# Autodesk Inventor assembly: ASY NVPH-400 shredder
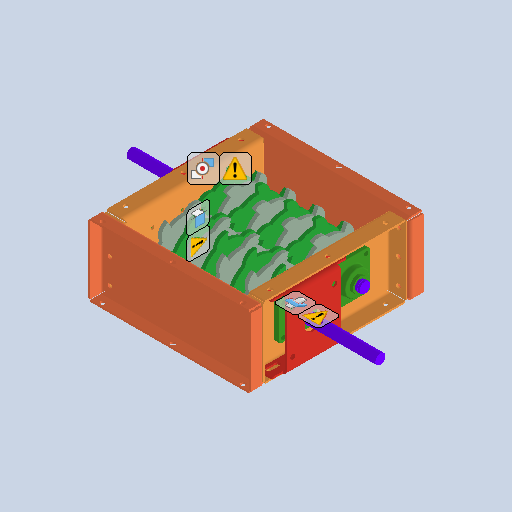
[picture p0: Inventor's stored thumbnail of the model, 512x512]
Saved by Autodesk Inventor 2025 (Build 290162010, 162A)
## iProperties
Created: 2024-12-13
Part Number: ASY NVPH-400 shredder
Document SubType Name: Assembly
Designer: user
Author: user
## Documents named in this file (12)
- C:\Users\pokla\Documents\Inventor\NDM-VOS_powder_hopper\ASY NVPH-400 shredder.iam
- C:\Users\pokla\Documents\Inventor\NDM-VOS_powder_hopper\ASY NVPH-200 shredder shaft full.iam
- C:\Users\pokla\Documents\Inventor\NDM-VOS_powder_hopper\NDM-VOS 111 sredder wall 1.ipt
- C:\Users\pokla\Documents\Inventor\NDM-VOS_powder_hopper\3d party\PCRV080-075SHFA_MS80B5\PCRV080-075SHFA_MS80B5\PCRV080-075SHFA_MS80B5.ipt
- C:\Users\pokla\Documents\Inventor\NDM-VOS_powder_hopper\NDM-VOS 112 sredder wall 2.ipt
- C:\Users\pokla\Documents\Inventor\NDM-VOS_powder_hopper\NDM-VOS dummy Disc Harrow Pillow block bearing mount Assembly.ipt
- C:\Users\DELL\YandexDisk-badmisterfox\домашниий пк\Inventor\Content Center Files\en-US\ISO 4017(1)\ISO 4017 - M12 x 35 - ISO.ipt
- C:\Users\pokla\Documents\Inventor\NDM-VOS_powder_hopper\NDM-VOS 116 engine plate.ipt
- C:\Users\DELL\YandexDisk-badmisterfox\домашниий пк\Inventor\Content Center Files\en-US\ISO 4017(1)\ISO 4017 - M12 x 40 - ISO.ipt
- C:\Users\pokla\Documents\Inventor\NDM-VOS_powder_hopper\NDM-VOS 161 harrow plate.ipt
- C:\Users\pokla\Documents\Inventor\NDM-VOS_powder_hopper\NDM-VOS 162 harrow plate 5.ipt
- C:\Users\DELL\YandexDisk-badmisterfox\домашниий пк\Inventor\Content Center Files\en-US\ISO 4017(1)\ISO 4017 - M12 x 25 - ISO.ipt
## Components (60 placed, 11 different names)
1. ASY NVPH-200 shredder shaft full:1 [sub-assembly] — Rotational:1, Mate:3
2. ASY NVPH-200 shredder shaft full:2 [sub-assembly] — Rotational:2, Mate:4
3. NDM-VOS 111 sredder wall 1:1 — Rigid:1, Rigid:3, Insert:13, Insert:14, Insert:15, Insert:17, Flush:1, Rigid:6, Rigid:7, Rotational:1, Rotational:13, Rotational:14, Slider:2, Rotational:15, Rotational:16
4. NDM-VOS 111 sredder wall 1:2 — Rigid:2, Insert:20, Insert:22, Insert:23, Insert:24, Rigid:8, Rigid:11, Rotational:2, Rotational:11, Rigid:12, Rigid:13, Rigid:14, Rigid:15, Rigid:16, Rigid:17, Rigid:18, Slider:1, Rigid:19, Rotational:12
5. PCRV080-075SHFA_MS80B5:1 — Rotational:17
6. PCRV080-075SHFA_MS80B5:2 — Rigid:20
7. NDM-VOS 112 sredder wall sub:1 — Rigid:1, Rigid:2, Insert:1, Insert:2, Insert:3, Insert:4, Insert:5, Insert:6, Insert:7, Insert:8, Insert:9, Insert:10, Insert:11, Insert:12, Mate:1, Mate:2
8. NDM-VOS 112 sredder wall sub:2 — Rigid:3, Insert:25, Insert:26, Insert:27, Insert:28, Insert:29, Insert:30, Insert:31, Insert:32, Insert:33, Insert:34, Insert:35, Insert:36
9. NDM-VOS dummy Disc Harrow Pillow block bearing mount Assembly:1 — Rigid:6
10. NDM-VOS dummy Disc Harrow Pillow block bearing mount Assembly:2 — Rigid:7
11. NDM-VOS dummy Disc Harrow Pillow block bearing mount Assembly:3 — Rigid:8
12. NDM-VOS dummy Disc Harrow Pillow block bearing mount Assembly:4 — Rigid:11
13. ISO 4017 M12 x 35:1 — Rotational:11
14. NDM-VOS 116 engine plate:1 — Slider:1, Mate:3, Rigid:20
15. ISO 4017 M12 x 40:37 — Rigid:12
16. ISO 4017 M12 x 40:38 — Rigid:13
17. ISO 4017 M12 x 40:39 — Rigid:14
18. ISO 4017 M12 x 40:40 — Rigid:15
19. ISO 4017 M12 x 40:41 — Rigid:16
20. ISO 4017 M12 x 40:42 — Rigid:17
21. ISO 4017 M12 x 40:43 — Rigid:18
22. NDM-VOS 161 harrow plate:1 — Rotational:15
23. NDM-VOS 162 harrow plate 5:1 — Rotational:16
24. NDM-VOS 116 engine plate:2 — Slider:2, Mate:4, Rotational:17
25. ISO 4017 M12 x 40:6 — Insert:1
26. ISO 4017 M12 x 40:11 — Insert:2
27. ISO 4017 M12 x 40:12 — Insert:3
28. ISO 4017 M12 x 40:13 — Insert:4
29. ISO 4017 M12 x 40:14 — Insert:5
30. ISO 4017 M12 x 40:15 — Insert:6
31. ISO 4017 M12 x 25:8 — Insert:7
32. ISO 4017 M12 x 25:4 — Insert:8
33. ISO 4017 M12 x 25:6 — Insert:9
34. ISO 4017 M12 x 25:5 — Insert:10
35. ISO 4017 M12 x 25:7 — Insert:11
36. ISO 4017 M12 x 25:9 — Insert:12
37. ISO 4017 M12 x 40:22 — Insert:13
38. ISO 4017 M12 x 40:23 — Insert:14
39. ISO 4017 M12 x 40:24 — Insert:15
40. ISO 4017 M12 x 40:9 — Rotational:14
41. ISO 4017 M12 x 40:10 — Insert:17
42. ISO 4017 M12 x 40:8 — Rotational:13
43. ISO 4017 M12 x 40:1 — Rotational:12
44. ISO 4017 M12 x 40:3 — Insert:20
45. ISO 4017 M12 x 40:5 — Rigid:19
46. ISO 4017 M12 x 40:25 — Insert:22
47. ISO 4017 M12 x 40:26 — Insert:23
48. ISO 4017 M12 x 40:27 — Insert:24
49. ISO 4017 M12 x 25:10 — Insert:25
50. ISO 4017 M12 x 25:12 — Insert:26
51. ISO 4017 M12 x 25:11 — Insert:27
52. ISO 4017 M12 x 25:3 — Insert:28
53. ISO 4017 M12 x 25:1 — Insert:29
54. ISO 4017 M12 x 25:2 — Insert:30
55. ISO 4017 M12 x 40:4 — Insert:31
56. ISO 4017 M12 x 40:7 — Insert:32
57. ISO 4017 M12 x 40:2 — Insert:33
58. ISO 4017 M12 x 40:34 — Insert:34
59. ISO 4017 M12 x 40:35 — Insert:35
60. ISO 4017 M12 x 40:36 — Insert:36
## Relationships (64: Insert 32, WeldJoint 16, RevoluteJoint 9, Mate 4, TranslationJoint 2, Flush 1)
- Rigid:1 [WeldJoint]: NDM-VOS 111 sredder wall 1:1 ↔ NDM-VOS 112 sredder wall sub:1
- Rigid:2 [WeldJoint]: NDM-VOS 111 sredder wall 1:2 ↔ NDM-VOS 112 sredder wall sub:1
- Rigid:3 [WeldJoint]: NDM-VOS 111 sredder wall 1:1 ↔ NDM-VOS 112 sredder wall sub:2
- Insert:1: NDM-VOS 112 sredder wall sub:1 ↔ ISO 4017 M12 x 40:6
- Insert:2: NDM-VOS 112 sredder wall sub:1 ↔ ISO 4017 M12 x 40:11
- Insert:3: NDM-VOS 112 sredder wall sub:1 ↔ ISO 4017 M12 x 40:12
- Insert:4: NDM-VOS 112 sredder wall sub:1 ↔ ISO 4017 M12 x 40:13
- Insert:5: NDM-VOS 112 sredder wall sub:1 ↔ ISO 4017 M12 x 40:14
- Insert:6: NDM-VOS 112 sredder wall sub:1 ↔ ISO 4017 M12 x 40:15
- Insert:7: NDM-VOS 112 sredder wall sub:1 ↔ ISO 4017 M12 x 25:8
- Insert:8: NDM-VOS 112 sredder wall sub:1 ↔ ISO 4017 M12 x 25:4
- Insert:9: NDM-VOS 112 sredder wall sub:1 ↔ ISO 4017 M12 x 25:6
- Insert:10: NDM-VOS 112 sredder wall sub:1 ↔ ISO 4017 M12 x 25:5
- Insert:11: NDM-VOS 112 sredder wall sub:1 ↔ ISO 4017 M12 x 25:7
- Insert:12: NDM-VOS 112 sredder wall sub:1 ↔ ISO 4017 M12 x 25:9
- Insert:13: NDM-VOS 111 sredder wall 1:1 ↔ ISO 4017 M12 x 40:22
- Insert:14: NDM-VOS 111 sredder wall 1:1 ↔ ISO 4017 M12 x 40:23
- Insert:15: NDM-VOS 111 sredder wall 1:1 ↔ ISO 4017 M12 x 40:24
- Insert:17: NDM-VOS 111 sredder wall 1:1 ↔ ISO 4017 M12 x 40:10
- Insert:20: NDM-VOS 111 sredder wall 1:2 ↔ ISO 4017 M12 x 40:3
- Insert:22: NDM-VOS 111 sredder wall 1:2 ↔ ISO 4017 M12 x 40:25
- Insert:23: NDM-VOS 111 sredder wall 1:2 ↔ ISO 4017 M12 x 40:26
- Insert:24: NDM-VOS 111 sredder wall 1:2 ↔ ISO 4017 M12 x 40:27
- Insert:25: NDM-VOS 112 sredder wall sub:2 ↔ ISO 4017 M12 x 25:10
- Insert:26: NDM-VOS 112 sredder wall sub:2 ↔ ISO 4017 M12 x 25:12
- Insert:27: NDM-VOS 112 sredder wall sub:2 ↔ ISO 4017 M12 x 25:11
- Insert:28: NDM-VOS 112 sredder wall sub:2 ↔ ISO 4017 M12 x 25:3
- Insert:29: NDM-VOS 112 sredder wall sub:2 ↔ ISO 4017 M12 x 25:1
- Insert:30: NDM-VOS 112 sredder wall sub:2 ↔ ISO 4017 M12 x 25:2
- Insert:31: NDM-VOS 112 sredder wall sub:2 ↔ ISO 4017 M12 x 40:4
- Insert:32: NDM-VOS 112 sredder wall sub:2 ↔ ISO 4017 M12 x 40:7
- Insert:33: NDM-VOS 112 sredder wall sub:2 ↔ ISO 4017 M12 x 40:2
- Insert:34: NDM-VOS 112 sredder wall sub:2 ↔ ISO 4017 M12 x 40:34
- Insert:35: NDM-VOS 112 sredder wall sub:2 ↔ ISO 4017 M12 x 40:35
- Insert:36: NDM-VOS 112 sredder wall sub:2 ↔ ISO 4017 M12 x 40:36
- Mate:1: NDM-VOS 112 sredder wall sub:1
- Mate:2: NDM-VOS 112 sredder wall sub:1
- Flush:1: NDM-VOS 111 sredder wall 1:1
- Rigid:6 [WeldJoint] (3 mm): NDM-VOS 111 sredder wall 1:1 ↔ NDM-VOS dummy Disc Harrow Pillow block bearing mount Assembly:1
- Rigid:7 [WeldJoint]: NDM-VOS 111 sredder wall 1:1 ↔ NDM-VOS dummy Disc Harrow Pillow block bearing mount Assembly:2
- Rigid:8 [WeldJoint] (-3 mm): NDM-VOS 111 sredder wall 1:2 ↔ NDM-VOS dummy Disc Harrow Pillow block bearing mount Assembly:3
- Rigid:11 [WeldJoint]: NDM-VOS 111 sredder wall 1:2 ↔ NDM-VOS dummy Disc Harrow Pillow block bearing mount Assembly:4
- Rotational:1 [RevoluteJoint] (-3 mm): ASY NVPH-200 shredder shaft full:1 ↔ NDM-VOS 111 sredder wall 1:1
- Rotational:2 [RevoluteJoint] (-3 mm): ASY NVPH-200 shredder shaft full:2 ↔ NDM-VOS 111 sredder wall 1:2
- Rotational:11 [RevoluteJoint]: NDM-VOS 111 sredder wall 1:2 ↔ ISO 4017 M12 x 35:1
- Rigid:12 [WeldJoint]: NDM-VOS 111 sredder wall 1:2 ↔ ISO 4017 M12 x 40:37
- Rigid:13 [WeldJoint]: NDM-VOS 111 sredder wall 1:2 ↔ ISO 4017 M12 x 40:38
- Rigid:14 [WeldJoint]: NDM-VOS 111 sredder wall 1:2 ↔ ISO 4017 M12 x 40:39
- Rigid:15 [WeldJoint]: NDM-VOS 111 sredder wall 1:2 ↔ ISO 4017 M12 x 40:40
- Rigid:16 [WeldJoint]: NDM-VOS 111 sredder wall 1:2 ↔ ISO 4017 M12 x 40:41
- Rigid:17 [WeldJoint]: NDM-VOS 111 sredder wall 1:2 ↔ ISO 4017 M12 x 40:42
- Rigid:18 [WeldJoint]: NDM-VOS 111 sredder wall 1:2 ↔ ISO 4017 M12 x 40:43
- Slider:1 [TranslationJoint] (-1 mm): NDM-VOS 111 sredder wall 1:2 ↔ NDM-VOS 116 engine plate:1
- Mate:3: ASY NVPH-200 shredder shaft full:1 ↔ NDM-VOS 116 engine plate:1
- Rigid:19 [WeldJoint] (-5 mm): NDM-VOS 111 sredder wall 1:2 ↔ ISO 4017 M12 x 40:5
- Rotational:12 [RevoluteJoint] (-5 mm): NDM-VOS 111 sredder wall 1:2 ↔ ISO 4017 M12 x 40:1
- Rigid:20 [WeldJoint]: PCRV080-075SHFA_MS80B5:2 ↔ NDM-VOS 116 engine plate:1
- Rotational:13 [RevoluteJoint] (-5 mm): NDM-VOS 111 sredder wall 1:1 ↔ ISO 4017 M12 x 40:8
- Rotational:14 [RevoluteJoint] (-5 mm): NDM-VOS 111 sredder wall 1:1 ↔ ISO 4017 M12 x 40:9
- Slider:2 [TranslationJoint] (-1 mm): NDM-VOS 111 sredder wall 1:1 ↔ NDM-VOS 116 engine plate:2
- Mate:4: ASY NVPH-200 shredder shaft full:2 ↔ NDM-VOS 116 engine plate:2
- Rotational:15 [RevoluteJoint]: NDM-VOS 111 sredder wall 1:1 ↔ NDM-VOS 161 harrow plate:1
- Rotational:16 [RevoluteJoint]: NDM-VOS 111 sredder wall 1:1 ↔ NDM-VOS 162 harrow plate 5:1
- Rotational:17 [RevoluteJoint]: PCRV080-075SHFA_MS80B5:1 ↔ NDM-VOS 116 engine plate:2
